# Autodesk Inventor assembly: car assembly
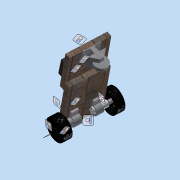
[picture p0: Inventor's stored thumbnail of the model, 180x180]
Saved by Autodesk Inventor 2015 (Build 190159000, 159)
## iProperties
Created: 2015-06-23
Part Number: car assembly
Document SubType Name: Assembly
Designer: Rahul
Author: Rahul
## Documents named in this file (11)
- C:\Users\Vincent\Desktop\car design\car assembly.iam
- C:\Users\Vincent\Desktop\car design\arduino.ipt
- C:\Users\Vincent\Desktop\car design\battery case.ipt
- C:\Users\Vincent\Desktop\car design\motor.ipt
- C:\Users\Vincent\Desktop\car design\wheel.ipt
- C:\Users\Vincent\Desktop\car design\base of car.ipt
- C:\Users\Vincent\Desktop\car design\caster wheel.ipt
- C:\Users\Vincent\Desktop\car design\base of car 2.ipt
- C:\Users\Vincent\Desktop\car design\motor mounts.ipt
- C:\Users\Vincent\Desktop\car design\breadboard lol.ipt
- C:\Users\Vincent\Desktop\car design\wheel connector.ipt
## Components (14 placed, 10 different names)
1. arduino:1 — Mate:22
2. battery case:1 — Mate:23
3. motor:2 — Insert:1, Tangent:1, Flush:7
4. wheel:1 — Mate:26, Mate:27
5. caster wheel:2 — Mate:17, Mate:21, Flush:6
6. base of car 2:1 — Mate:17, Mate:20, Mate:21, Flush:3, Flush:6, Mate:23
7. wheel:2 — Mate:28, Mate:29
8. motor mounts:1 — Mate:24, Tangent:2, Flush:9
9. motor mounts:2 — Mate:25, Tangent:1
10. breadboard lol:1 — Mate:18
11. base of car:1 — Mate:18, Mate:20, Flush:3, Mate:22, Mate:24, Mate:25, Flush:7, Flush:8, Flush:9
12. wheel connector:1 — Insert:1, Mate:26, Mate:27
13. motor:3 — Tangent:2, Flush:8, Insert:2
14. wheel connector:2 — Mate:28, Mate:29, Insert:2
## Relationships (21: Mate 12, Flush 5, Insert 2, Tangent 2)
- Mate:17: caster wheel:2 ↔ base of car 2:1
- Mate:18: breadboard lol:1 ↔ base of car:1
- Mate:20: base of car 2:1 ↔ base of car:1
- Mate:21: caster wheel:2 ↔ base of car 2:1
- Flush:3: base of car 2:1 ↔ base of car:1
- Flush:6: caster wheel:2 ↔ base of car 2:1
- Insert:1: motor:2 ↔ wheel connector:1
- Mate:22: arduino:1 ↔ base of car:1
- Mate:23: battery case:1 ↔ base of car 2:1
- Mate:24: motor mounts:1 ↔ base of car:1
- Mate:25: motor mounts:2 ↔ base of car:1
- Tangent:1: motor:2 ↔ motor mounts:2
- Flush:7: motor:2 ↔ base of car:1
- Mate:26: wheel:1 ↔ wheel connector:1
- Mate:27: wheel:1 ↔ wheel connector:1
- Tangent:2: motor mounts:1 ↔ motor:3
- Flush:8: base of car:1 ↔ motor:3
- Mate:28: wheel:2 ↔ wheel connector:2
- Mate:29: wheel:2 ↔ wheel connector:2
- Insert:2: motor:3 ↔ wheel connector:2
- Flush:9: motor mounts:1 ↔ base of car:1
